# Autodesk Inventor assembly: Drive Beginnings
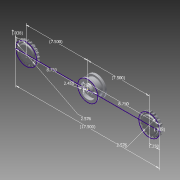
[picture p0: Inventor's stored thumbnail of the model, 180x180]
Saved by Autodesk Inventor 2015 (Build 190159000, 159)
## iProperties
Created: 2015-10-02
Part Number: Drive Beginnings
Document SubType Name: Assembly
Designer: alhohbein
Author: alhohbein
## Documents named in this file (4)
- U:\Drive Beginnings.iam
- U:\tetrix_736468_tt_wheel_2012.ipt
- U:\Tetrix tread sprocket.ipt
- U:\Drive basic measurements.ipt
## Components (4 placed, 3 different names)
1. tetrix_736468_tt_wheel_2012:1 — Mate:1
2. Tetrix tread sprocket:1 — Mate:2
3. Tetrix tread sprocket:2 — Mate:3
4. Drive basic measurements:1 — Mate:1, Mate:2, Mate:3
## Relationships (3: Mate 3)
- Mate:1: tetrix_736468_tt_wheel_2012:1 ↔ Drive basic measurements:1
- Mate:2: Tetrix tread sprocket:1 ↔ Drive basic measurements:1
- Mate:3: Tetrix tread sprocket:2 ↔ Drive basic measurements:1
